# Autodesk Inventor assembly: Podstawa
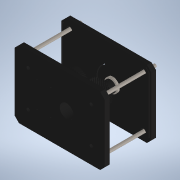
[picture p0: Inventor's stored thumbnail of the model, 180x180]
Saved by Autodesk Inventor 2021 (Build 250183000, 183)
## iProperties
Created: 2021-07-30
Part Number: Podstawa
Document SubType Name: Assembly
Designer: Janusz
Author: Janusz
Revision Number: ANY
## Documents named in this file (11)
- D:\ROBOT\Podstawa.iam
- D:\ROBOT\Podstawa_Dolna_cz©.ipt
- D:\ROBOT\Podstawa_G¢rna_cz©.ipt
- D:\ROBOT\rod_8mm_120 mm.ipt
- D:\ROBOT\bering_osiowy_17x30x9.ipt
- D:\ROBOT\Zêbatka_podstawa_walek_ISO - RH Helical gear 1M 35T 45HA 20PA 15FW ---35C20H34L8.0N.ipt
- D:\ROBOT\Zêbatka_podstawa_silnik_ISO - RH Helical gear 1M 35T 45HA 20PA 10FW ---35B30H20L5.0N.ipt
- D:\ROBOT\silnik_podstawy_z_mocowaniem.iam
- D:\ROBOT\Obudowa_podstawy.ipt
- D:\ROBOT\bering.ipt
- D:\ROBOT\ISO 10642 - M3 x 10 - 10N_ISO 10642 - M3 x 10 - 10N.ipt
## Components (18 placed, 18 different names)
1. Podstawa_Dolna_cz©_78 — Wstawiające:1, Wstawiające:2, Wstawiające:3, Wstawiające:4
2. Podstawa_G¢rna_cz©_79 — Zestawiające:1, Zestawiające:2
3. rod_8mm_120 mm_80 — Wstawiające:2
4. rod_8mm_120 mm_81 — Wstawiające:4
5. rod_8mm_120 mm_82 — Wstawiające:3, Zestawiające:2
6. rod_8mm_120 mm_83 — Wstawiające:1, Zestawiające:1
7. bering_osiowy_17x30x9_84
8. bering_osiowy_17x30x9_85
9. bering_osiowy_17x30x9_86
10. bering_osiowy_17x30x9_87
11. Zêbatka_podstawa_walek_ISO - RH Helical gear 1M 35T 45HA 20PA 15FW ---35C20H34L8.0N_88
12. Zêbatka_podstawa_silnik_ISO - RH Helical gear 1M 35T 45HA 20PA 10FW ---35B30H20L5.0N_89
13. silnik_podstawy_z_mocowaniem_90 [sub-assembly]
14. Obudowa_podstawy_95
15. bering_96
16. bering_97
17. ISO 10642 - M3 x 10 - 10N_ISO 10642 - M3 x 10 - 10N_98
18. ISO 10642 - M3 x 10 - 10N_ISO 10642 - M3 x 10 - 10N_99
## Relationships (6: Insert 4, Mate 2)
- Wstawiające:1 [Insert]: Podstawa_Dolna_cz©_78 ↔ rod_8mm_120 mm_83
- Wstawiające:2 [Insert]: Podstawa_Dolna_cz©_78 ↔ rod_8mm_120 mm_80
- Wstawiające:3 [Insert]: Podstawa_Dolna_cz©_78 ↔ rod_8mm_120 mm_82
- Wstawiające:4 [Insert]: Podstawa_Dolna_cz©_78 ↔ rod_8mm_120 mm_81
- Zestawiające:1 [Mate]: Podstawa_G¢rna_cz©_79 ↔ rod_8mm_120 mm_83
- Zestawiające:2 [Mate]: Podstawa_G¢rna_cz©_79 ↔ rod_8mm_120 mm_82
